# Autodesk Inventor assembly: ClawAssembly
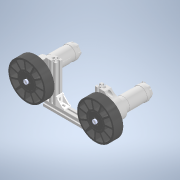
[picture p0: Inventor's stored thumbnail of the model, 180x180]
Saved by Autodesk Inventor 2020.2 (Build 242310000, 310)
## iProperties
Created: 2020-01-29
Part Number: ClawAssembly
Document SubType Name: Assembly
Designer: Jimmy
Author: Jimmy
## Documents named in this file (9)
- C:\Users\AOFUser\Desktop\Robotics\ClawAssembly.iam
- C:\Users\AOFUser\Desktop\Robotics\RevHexMotor\RevHexMotor.iam
- C:\Users\AOFUser\Desktop\Robotics\AndymarkCompliantWheels\CompliantWheel.iam
- C:\Users\AOFUser\Desktop\Robotics\Motor Mount vCAD.ipt
- C:\Users\AOFUser\Desktop\Robotics\ShaftCollar.ipt
- C:\Users\AOFUser\Desktop\Robotics\HexHub.ipt
- C:\Users\AOFUser\Desktop\Robotics\Extrusions\4in.ipt
- C:\Users\AOFUser\Desktop\Robotics\CornerBracket.ipt
- C:\Users\AOFUser\Desktop\Robotics\Extrusions\7in.ipt
## Components (15 placed, 8 different names)
1. RevHexMotor:2 [sub-assembly] — Insert:3, Insert:4, Mate:1, Mate:2, Mate:3
2. CompliantWheel:1 [sub-assembly] — Insert:5, Insert:6, Insert:7
3. Motor Mount vCAD:1 — Insert:3, Insert:4, Mate:7, Flush:2, Flush:9
4. ShaftCollar:1 — Insert:7
5. HexHub:1 — Insert:5, Insert:6, Mate:1, Mate:2, Mate:3
6. RevHexMotor:3 [sub-assembly] — Insert:13, Insert:14
7. CompliantWheel:2 [sub-assembly]
8. Motor Mount vCAD:2 — Flush:3, Mate:8, Flush:4, Insert:13, Insert:14
9. ShaftCollar:2
10. HexHub:2
11. 4in:1 — Mate:7, Flush:2, Flush:9, Mate:12, Flush:12, Flush:13
12. 4in:2 — Flush:3, Mate:8, Flush:4, Mate:9, Flush:5, Flush:6
13. CornerBracket:1 — Mate:9, Flush:5, Flush:6, Flush:7, Mate:10, Flush:8
14. CornerBracket:5 — Flush:10, Flush:11, Mate:11, Mate:12, Flush:12, Flush:13
15. 7in:1 — Flush:7, Mate:10, Flush:8, Flush:10, Flush:11, Mate:11
## Relationships (34: Mate 12, Flush 12, Insert 10)
- Insert:3: RevHexMotor:2 ↔ Motor Mount vCAD:1
- Insert:4: RevHexMotor:2 ↔ Motor Mount vCAD:1
- Insert:5: CompliantWheel:1 ↔ HexHub:1
- Insert:6: CompliantWheel:1 ↔ HexHub:1
- Mate:1: RevHexMotor:2 ↔ HexHub:1
- Mate:2: RevHexMotor:2 ↔ HexHub:1
- Mate:3: RevHexMotor:2 ↔ HexHub:1
- Insert:7: CompliantWheel:1 ↔ ShaftCollar:1
- [Insert]: CompliantWheel:2 ↔ HexHub:2
- [Insert]: CompliantWheel:2 ↔ HexHub:2
- [Mate]: RevHexMotor:3 ↔ HexHub:2
- [Mate]: RevHexMotor:3 ↔ HexHub:2
- [Mate]: RevHexMotor:3 ↔ HexHub:2
- [Insert]: CompliantWheel:2 ↔ ShaftCollar:2
- Mate:7: Motor Mount vCAD:1 ↔ 4in:1
- Flush:2: Motor Mount vCAD:1 ↔ 4in:1
- Flush:3: Motor Mount vCAD:2 ↔ 4in:2
- Mate:8: Motor Mount vCAD:2 ↔ 4in:2
- Flush:4: Motor Mount vCAD:2 ↔ 4in:2
- Mate:9: 4in:2 ↔ CornerBracket:1
- Flush:5: 4in:2 ↔ CornerBracket:1
- Flush:6: 4in:2 ↔ CornerBracket:1
- Flush:7: CornerBracket:1 ↔ 7in:1
- Mate:10: CornerBracket:1 ↔ 7in:1
- Flush:8 (34.925 mm): CornerBracket:1 ↔ 7in:1
- Insert:13: RevHexMotor:3 ↔ Motor Mount vCAD:2
- Insert:14: RevHexMotor:3 ↔ Motor Mount vCAD:2
- Flush:9: Motor Mount vCAD:1 ↔ 4in:1
- Flush:10: CornerBracket:5 ↔ 7in:1
- Flush:11 (34.925 mm): CornerBracket:5 ↔ 7in:1
- Mate:11: CornerBracket:5 ↔ 7in:1
- Mate:12: 4in:1 ↔ CornerBracket:5
- Flush:12: 4in:1 ↔ CornerBracket:5
- Flush:13: 4in:1 ↔ CornerBracket:5
## Named parameters: d43_d37 = 0 mm, d44_d38 = 0 mm, d45_d39 = 0 mm, d46_d40 = 0 mm, d47_d42 = 0 mm, d50_d36 = 0 mm
